# Autodesk Inventor assembly: rackAssembly
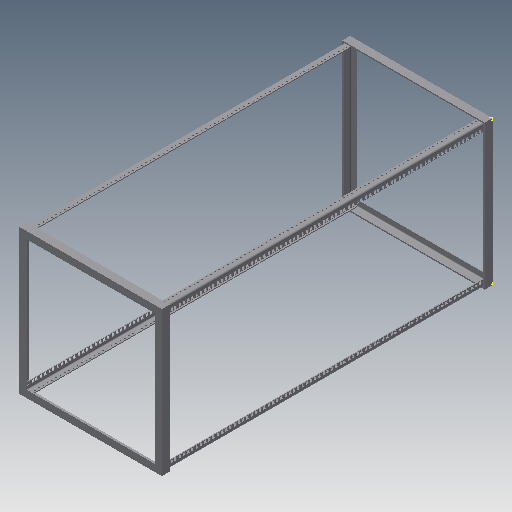
[picture p0: Inventor's stored thumbnail of the model, 512x512]
Saved by Autodesk Inventor 2017 (Build 210142000, 142)
## iProperties
Created: 2016-08-03
Part Number: rackAssembly
Document SubType Name: Assembly
Designer: Zuhra Abdurashidova
Author: Zuhra Abdurashidova
## Documents named in this file (4)
- C:\Users\krosie\Google Drive\HERA\hera-cad\Node\rackAssembly.iam
- C:\Users\krosie\Google Drive\HERA\hera-cad\Node\squareHoleRail20U.ipt
- C:\Users\krosie\Google Drive\HERA\hera-cad\Node\squareHoleRail20Umirror.ipt
- C:\Users\krosie\Google Drive\HERA\hera-cad\Node\rackBase.ipt
## Components (6 placed, 3 different names)
1. squareHoleRail20U:2 — Mate:1, Mate:2, Mate:3, Mate:13, Mate:16
2. squareHoleRail20Umirror:1 — Mate:4, Mate:5, Mate:6
3. squareHoleRail20Umirror:2 — Mate:10, Mate:11, Mate:12, Mate:14, Mate:15
4. rackBase:1 — Mate:1, Mate:2, Mate:3, Mate:4, Mate:5, Mate:6, Mate:7, Mate:8, Mate:9, Mate:10, Mate:11, Mate:12
5. rackBase:2 — Mate:13, Mate:14, Mate:15, Mate:16
6. squareHoleRail20U:3 — Mate:7, Mate:8, Mate:9
## Relationships (16: Mate 16)
- Mate:1: squareHoleRail20U:2 ↔ rackBase:1
- Mate:2: squareHoleRail20U:2 ↔ rackBase:1
- Mate:3: squareHoleRail20U:2 ↔ rackBase:1
- Mate:4: squareHoleRail20Umirror:1 ↔ rackBase:1
- Mate:5: squareHoleRail20Umirror:1 ↔ rackBase:1
- Mate:6: squareHoleRail20Umirror:1 ↔ rackBase:1
- Mate:7: rackBase:1 ↔ squareHoleRail20U:3
- Mate:8: rackBase:1 ↔ squareHoleRail20U:3
- Mate:9: rackBase:1 ↔ squareHoleRail20U:3
- Mate:10: squareHoleRail20Umirror:2 ↔ rackBase:1
- Mate:11: squareHoleRail20Umirror:2 ↔ rackBase:1
- Mate:12: squareHoleRail20Umirror:2 ↔ rackBase:1
- Mate:13: squareHoleRail20U:2 ↔ rackBase:2
- Mate:14: squareHoleRail20Umirror:2 ↔ rackBase:2
- Mate:15: squareHoleRail20Umirror:2 ↔ rackBase:2
- Mate:16: squareHoleRail20U:2 ↔ rackBase:2
